# Autodesk Inventor assembly: CHIP_CONTAINER
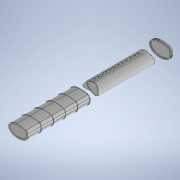
[picture p0: Inventor's stored thumbnail of the model, 180x180]
Saved by Autodesk Inventor 2022 (Build 260153070, 153G)
## iProperties
Created: 2022-04-01
Part Number: CHIP_CONTAINER
Document SubType Name: Assembly
Designer: a laptop
Author: a laptop
## Documents named in this file (5)
- C:\Users\a laptop\Desktop\CADTable_2022_Project\CHIP_CONTAINER.iam
- C:\Users\a laptop\Desktop\CADTable_2022_Project\Container_Design1.ipt
- C:\Users\a laptop\Desktop\CADTable_2022_Project\CHIP.ipt
- C:\Users\a laptop\Desktop\CADTable_2022_Project\chip_holder_V2.ipt
- C:\Users\a laptop\Desktop\CADTable_2022_Project\chip_lid.ipt
## Components (103 placed, 4 different names)
1. Container_Design1:1 — Mate:3, Angle:2, Mate:4, Mate:5, Angle:3, Mate:7
2. chip_holder_V2:1 — Mate:1, Angle:1, Mate:2, Mate:3, Angle:2, Mate:4
3. chip_lid:1 — Mate:5, Angle:3, Mate:7
4. CHIP:1 — Mate:1, Angle:1, Mate:2
5. CHIP:2
6. CHIP:3
7. CHIP:4
8. CHIP:5
9. CHIP:6
10. CHIP:7
11. CHIP:8
12. CHIP:9
13. CHIP:10
14. CHIP:11
15. CHIP:12
16. CHIP:13
17. CHIP:14
18. CHIP:15
19. CHIP:16
20. CHIP:17
21. CHIP:18
22. CHIP:19
23. CHIP:20
24. CHIP:21
25. CHIP:22
26. CHIP:23
27. CHIP:24
28. CHIP:25
29. CHIP:26
30. CHIP:27
31. CHIP:28
32. CHIP:29
33. CHIP:30
34. CHIP:31
35. CHIP:32
36. CHIP:33
37. CHIP:34
38. CHIP:35
39. CHIP:36
40. CHIP:37
41. CHIP:38
42. CHIP:39
43. CHIP:40
44. CHIP:41
45. CHIP:42
46. CHIP:43
47. CHIP:44
48. CHIP:45
49. CHIP:46
50. CHIP:47
51. CHIP:48
52. CHIP:49
53. CHIP:50
54. CHIP:51
55. CHIP:52
56. CHIP:53
57. CHIP:54
58. CHIP:55
59. CHIP:56
60. CHIP:57
61. CHIP:58
62. CHIP:59
63. CHIP:60
64. CHIP:61
65. CHIP:62
66. CHIP:63
67. CHIP:64
68. CHIP:65
69. CHIP:66
70. CHIP:67
71. CHIP:68
72. CHIP:69
73. CHIP:70
74. CHIP:71
75. CHIP:72
76. CHIP:73
77. CHIP:74
78. CHIP:75
79. CHIP:76
80. CHIP:77
81. CHIP:78
82. CHIP:79
83. CHIP:80
84. CHIP:81
85. CHIP:82
86. CHIP:83
87. CHIP:84
88. CHIP:85
89. CHIP:86
90. CHIP:87
91. CHIP:88
92. CHIP:89
93. CHIP:90
94. CHIP:91
95. CHIP:92
96. CHIP:93
97. CHIP:94
98. CHIP:95
99. CHIP:96
100. CHIP:97
101. CHIP:98
102. CHIP:99
103. CHIP:100
## Component patterns: (100 elements, first: CHIP:1)
## Relationships (9: Mate 6, Angle 3)
- Mate:1: chip_holder_V2:1 ↔ CHIP:1
- Angle:1 (0 deg): chip_holder_V2:1 ↔ CHIP:1
- Mate:2: chip_holder_V2:1 ↔ CHIP:1
- Mate:3: Container_Design1:1 ↔ chip_holder_V2:1
- Angle:2 (0 deg): Container_Design1:1 ↔ chip_holder_V2:1
- Mate:4: Container_Design1:1 ↔ chip_holder_V2:1
- Mate:5: Container_Design1:1 ↔ chip_lid:1
- Angle:3 (0 deg): Container_Design1:1 ↔ chip_lid:1
- Mate:7: Container_Design1:1 ↔ chip_lid:1
